# Autodesk Inventor assembly: Grupo_cortadora_MIR
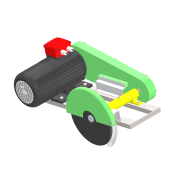
[picture p0: Inventor's stored thumbnail of the model, 180x180]
Saved by Autodesk Inventor 2021 (Build 250183000, 183)
## iProperties
Created: 2021-04-30
Part Number: Grupo_cortadora_MIR
Document SubType Name: Assembly
Designer: maaro
Sending System: Autodesk Translation Framework
Major Version: 7.0
Minor Version: 0.0
Format Version: 0.0
Product Id: Autodesk Translation Framework
Author: Admin
## Documents named in this file (84)
- C:\Users\maaro\Documents\UNAL\Automatización de Procesos de Manufactura\Github\Proyecto_APM\CADs estaciones a automatizar\Estación corte\Grupo_cortadora_MIR.iam
- C:\Users\maaro\Documents\UNAL\Automatización de Procesos de Manufactura\Github\Proyecto_APM\CADs estaciones a automatizar\Estación corte\Grupo_cortadora_MIR.ipt
- C:\Users\maaro\Documents\UNAL\Automatización de Procesos de Manufactura\Github\Proyecto_APM\CADs estaciones a automatizar\Estación corte\Grupo_cortadora_1_MIR.ipt
- C:\Users\maaro\Documents\UNAL\Automatización de Procesos de Manufactura\Github\Proyecto_APM\CADs estaciones a automatizar\Estación corte\Grupo_cortadora_2_MIR.ipt
- C:\Users\maaro\Documents\UNAL\Automatización de Procesos de Manufactura\Github\Proyecto_APM\CADs estaciones a automatizar\Estación corte\Grupo_cortadora_3_MIR.ipt
- C:\Users\maaro\Documents\UNAL\Automatización de Procesos de Manufactura\Github\Proyecto_APM\CADs estaciones a automatizar\Estación corte\Grupo_cortadora_4_MIR.ipt
- C:\Users\maaro\Documents\UNAL\Automatización de Procesos de Manufactura\Github\Proyecto_APM\CADs estaciones a automatizar\Estación corte\Grupo_cortadora_5_MIR.ipt
- C:\Users\maaro\Documents\UNAL\Automatización de Procesos de Manufactura\Github\Proyecto_APM\CADs estaciones a automatizar\Estación corte\Grupo_cortadora_6_MIR.ipt
- C:\Users\maaro\Documents\UNAL\Automatización de Procesos de Manufactura\Github\Proyecto_APM\CADs estaciones a automatizar\Estación corte\Grupo_cortadora_7_MIR.ipt
- C:\Users\maaro\Documents\UNAL\Automatización de Procesos de Manufactura\Github\Proyecto_APM\CADs estaciones a automatizar\Estación corte\Grupo_cortadora_8_MIR.ipt
- C:\Users\maaro\Documents\UNAL\Automatización de Procesos de Manufactura\Github\Proyecto_APM\CADs estaciones a automatizar\Estación corte\Grupo_cortadora_9_MIR.ipt
- C:\Users\maaro\Documents\UNAL\Automatización de Procesos de Manufactura\Github\Proyecto_APM\CADs estaciones a automatizar\Estación corte\Grupo_cortadora_10_MIR.ipt
- C:\Users\maaro\Documents\UNAL\Automatización de Procesos de Manufactura\Github\Proyecto_APM\CADs estaciones a automatizar\Estación corte\Grupo_cortadora_11_MIR.ipt
- C:\Users\maaro\Documents\UNAL\Automatización de Procesos de Manufactura\Github\Proyecto_APM\CADs estaciones a automatizar\Estación corte\Grupo_cortadora_12_MIR.ipt
- C:\Users\maaro\Documents\UNAL\Automatización de Procesos de Manufactura\Github\Proyecto_APM\CADs estaciones a automatizar\Estación corte\Grupo_cortadora_13_MIR.ipt
- C:\Users\maaro\Documents\UNAL\Automatización de Procesos de Manufactura\Github\Proyecto_APM\CADs estaciones a automatizar\Estación corte\Grupo_cortadora_17_MIR.ipt
- C:\Users\maaro\Documents\UNAL\Automatización de Procesos de Manufactura\Github\Proyecto_APM\CADs estaciones a automatizar\Estación corte\Grupo_cortadora_18_MIR.ipt
- C:\Users\maaro\Documents\UNAL\Automatización de Procesos de Manufactura\Github\Proyecto_APM\CADs estaciones a automatizar\Estación corte\Grupo_cortadora_20_MIR.ipt
- C:\Users\maaro\Documents\UNAL\Automatización de Procesos de Manufactura\Github\Proyecto_APM\CADs estaciones a automatizar\Estación corte\Grupo_cortadora_21_MIR.ipt
- C:\Users\maaro\Documents\UNAL\Automatización de Procesos de Manufactura\Github\Proyecto_APM\CADs estaciones a automatizar\Estación corte\Grupo_cortadora_22_MIR.ipt
- C:\Users\maaro\Documents\UNAL\Automatización de Procesos de Manufactura\Github\Proyecto_APM\CADs estaciones a automatizar\Estación corte\Grupo_cortadora_23_MIR.ipt
- C:\Users\maaro\Documents\UNAL\Automatización de Procesos de Manufactura\Github\Proyecto_APM\CADs estaciones a automatizar\Estación corte\Grupo_cortadora_24_MIR.ipt
- C:\Users\maaro\Documents\UNAL\Automatización de Procesos de Manufactura\Github\Proyecto_APM\CADs estaciones a automatizar\Estación corte\Grupo_cortadora_25_MIR.ipt
- C:\Users\maaro\Documents\UNAL\Automatización de Procesos de Manufactura\Github\Proyecto_APM\CADs estaciones a automatizar\Estación corte\Grupo_cortadora_26_MIR.ipt
- C:\Users\maaro\Documents\UNAL\Automatización de Procesos de Manufactura\Github\Proyecto_APM\CADs estaciones a automatizar\Estación corte\Grupo_cortadora_27_MIR.ipt
- C:\Users\maaro\Documents\UNAL\Automatización de Procesos de Manufactura\Github\Proyecto_APM\CADs estaciones a automatizar\Estación corte\Grupo_cortadora_28_MIR.ipt
- C:\Users\maaro\Documents\UNAL\Automatización de Procesos de Manufactura\Github\Proyecto_APM\CADs estaciones a automatizar\Estación corte\Grupo_cortadora_29_MIR.ipt
- C:\Users\maaro\Documents\UNAL\Automatización de Procesos de Manufactura\Github\Proyecto_APM\CADs estaciones a automatizar\Estación corte\Grupo_cortadora_30_MIR.ipt
- C:\Users\maaro\Documents\UNAL\Automatización de Procesos de Manufactura\Github\Proyecto_APM\CADs estaciones a automatizar\Estación corte\Grupo_cortadora_31_MIR.ipt
- C:\Users\maaro\Documents\UNAL\Automatización de Procesos de Manufactura\Github\Proyecto_APM\CADs estaciones a automatizar\Estación corte\Grupo_cortadora_32_MIR.ipt
- C:\Users\maaro\Documents\UNAL\Automatización de Procesos de Manufactura\Github\Proyecto_APM\CADs estaciones a automatizar\Estación corte\Grupo_cortadora_33_MIR.ipt
- C:\Users\maaro\Documents\UNAL\Automatización de Procesos de Manufactura\Github\Proyecto_APM\CADs estaciones a automatizar\Estación corte\Grupo_cortadora_34_MIR.ipt
- C:\Users\maaro\Documents\UNAL\Automatización de Procesos de Manufactura\Github\Proyecto_APM\CADs estaciones a automatizar\Estación corte\Grupo_cortadora_35_MIR.ipt
- C:\Users\maaro\Documents\UNAL\Automatización de Procesos de Manufactura\Github\Proyecto_APM\CADs estaciones a automatizar\Estación corte\Grupo_cortadora_36_MIR.ipt
- C:\Users\maaro\Documents\UNAL\Automatización de Procesos de Manufactura\Github\Proyecto_APM\CADs estaciones a automatizar\Estación corte\Grupo_cortadora_37_MIR.ipt
- C:\Users\maaro\Documents\UNAL\Automatización de Procesos de Manufactura\Github\Proyecto_APM\CADs estaciones a automatizar\Estación corte\Grupo_cortadora_38_MIR.ipt
- C:\Users\maaro\Documents\UNAL\Automatización de Procesos de Manufactura\Github\Proyecto_APM\CADs estaciones a automatizar\Estación corte\Grupo_cortadora_39_MIR.ipt
- C:\Users\maaro\Documents\UNAL\Automatización de Procesos de Manufactura\Github\Proyecto_APM\CADs estaciones a automatizar\Estación corte\Grupo_cortadora_40_MIR.ipt
- C:\Users\maaro\Documents\UNAL\Automatización de Procesos de Manufactura\Github\Proyecto_APM\CADs estaciones a automatizar\Estación corte\Grupo_cortadora_41_MIR.ipt
- C:\Users\maaro\Documents\UNAL\Automatización de Procesos de Manufactura\Github\Proyecto_APM\CADs estaciones a automatizar\Estación corte\Grupo_cortadora_42_MIR.ipt
- C:\Users\maaro\Documents\UNAL\Automatización de Procesos de Manufactura\Github\Proyecto_APM\CADs estaciones a automatizar\Estación corte\Grupo_cortadora_43_MIR.ipt
- C:\Users\maaro\Documents\UNAL\Automatización de Procesos de Manufactura\Github\Proyecto_APM\CADs estaciones a automatizar\Estación corte\Grupo_cortadora_44_MIR.ipt
- C:\Users\maaro\Documents\UNAL\Automatización de Procesos de Manufactura\Github\Proyecto_APM\CADs estaciones a automatizar\Estación corte\Grupo_cortadora_45_MIR.ipt
- C:\Users\maaro\Documents\UNAL\Automatización de Procesos de Manufactura\Github\Proyecto_APM\CADs estaciones a automatizar\Estación corte\Grupo_cortadora_46_MIR.ipt
- C:\Users\maaro\Documents\UNAL\Automatización de Procesos de Manufactura\Github\Proyecto_APM\CADs estaciones a automatizar\Estación corte\Grupo_cortadora_47_MIR.ipt
- C:\Users\maaro\Documents\UNAL\Automatización de Procesos de Manufactura\Github\Proyecto_APM\CADs estaciones a automatizar\Estación corte\Grupo_cortadora_48_MIR.ipt
- C:\Users\maaro\Documents\UNAL\Automatización de Procesos de Manufactura\Github\Proyecto_APM\CADs estaciones a automatizar\Estación corte\Grupo_cortadora_49_MIR.ipt
- C:\Users\maaro\Documents\UNAL\Automatización de Procesos de Manufactura\Github\Proyecto_APM\CADs estaciones a automatizar\Estación corte\Grupo_cortadora_50_MIR.ipt
- C:\Users\maaro\Documents\UNAL\Automatización de Procesos de Manufactura\Github\Proyecto_APM\CADs estaciones a automatizar\Estación corte\Grupo_cortadora_51_MIR.ipt
- C:\Users\maaro\Documents\UNAL\Automatización de Procesos de Manufactura\Github\Proyecto_APM\CADs estaciones a automatizar\Estación corte\Grupo_cortadora_52_MIR.ipt
- C:\Users\maaro\Documents\UNAL\Automatización de Procesos de Manufactura\Github\Proyecto_APM\CADs estaciones a automatizar\Estación corte\Grupo_cortadora_53_MIR.ipt
- C:\Users\maaro\Documents\UNAL\Automatización de Procesos de Manufactura\Github\Proyecto_APM\CADs estaciones a automatizar\Estación corte\Grupo_cortadora_54_MIR.ipt
- C:\Users\maaro\Documents\UNAL\Automatización de Procesos de Manufactura\Github\Proyecto_APM\CADs estaciones a automatizar\Estación corte\Grupo_cortadora_55_MIR.ipt
- C:\Users\maaro\Documents\UNAL\Automatización de Procesos de Manufactura\Github\Proyecto_APM\CADs estaciones a automatizar\Estación corte\Grupo_cortadora_56_MIR.ipt
- C:\Users\maaro\Documents\UNAL\Automatización de Procesos de Manufactura\Github\Proyecto_APM\CADs estaciones a automatizar\Estación corte\Grupo_cortadora_57_MIR.ipt
- C:\Users\maaro\Documents\UNAL\Automatización de Procesos de Manufactura\Github\Proyecto_APM\CADs estaciones a automatizar\Estación corte\Grupo_cortadora_58_MIR.ipt
- C:\Users\maaro\Documents\UNAL\Automatización de Procesos de Manufactura\Github\Proyecto_APM\CADs estaciones a automatizar\Estación corte\Grupo_cortadora_59_MIR.ipt
- C:\Users\maaro\Documents\UNAL\Automatización de Procesos de Manufactura\Github\Proyecto_APM\CADs estaciones a automatizar\Estación corte\Grupo_cortadora_60_MIR.ipt
- C:\Users\maaro\Documents\UNAL\Automatización de Procesos de Manufactura\Github\Proyecto_APM\CADs estaciones a automatizar\Estación corte\Grupo_cortadora_61_MIR.ipt
- C:\Users\maaro\Documents\UNAL\Automatización de Procesos de Manufactura\Github\Proyecto_APM\CADs estaciones a automatizar\Estación corte\Grupo_cortadora_62_MIR.ipt
- C:\Users\maaro\Documents\UNAL\Automatización de Procesos de Manufactura\Github\Proyecto_APM\CADs estaciones a automatizar\Estación corte\Grupo_cortadora_63_MIR.ipt
- C:\Users\maaro\Documents\UNAL\Automatización de Procesos de Manufactura\Github\Proyecto_APM\CADs estaciones a automatizar\Estación corte\Grupo_cortadora_64_MIR.ipt
- C:\Users\maaro\Documents\UNAL\Automatización de Procesos de Manufactura\Github\Proyecto_APM\CADs estaciones a automatizar\Estación corte\Grupo_cortadora_65_MIR.ipt
- C:\Users\maaro\Documents\UNAL\Automatización de Procesos de Manufactura\Github\Proyecto_APM\CADs estaciones a automatizar\Estación corte\Grupo_cortadora_66_MIR.ipt
- C:\Users\maaro\Documents\UNAL\Automatización de Procesos de Manufactura\Github\Proyecto_APM\CADs estaciones a automatizar\Estación corte\Grupo_cortadora_67_MIR.ipt
- C:\Users\maaro\Documents\UNAL\Automatización de Procesos de Manufactura\Github\Proyecto_APM\CADs estaciones a automatizar\Estación corte\Grupo_cortadora_68_MIR.ipt
- C:\Users\maaro\Documents\UNAL\Automatización de Procesos de Manufactura\Github\Proyecto_APM\CADs estaciones a automatizar\Estación corte\Grupo_cortadora_69_MIR.ipt
- C:\Users\maaro\Documents\UNAL\Automatización de Procesos de Manufactura\Github\Proyecto_APM\CADs estaciones a automatizar\Estación corte\Grupo_cortadora_70_MIR.ipt
- C:\Users\maaro\Documents\UNAL\Automatización de Procesos de Manufactura\Github\Proyecto_APM\CADs estaciones a automatizar\Estación corte\Grupo_cortadora_71_MIR.ipt
- C:\Users\maaro\Documents\UNAL\Automatización de Procesos de Manufactura\Github\Proyecto_APM\CADs estaciones a automatizar\Estación corte\Grupo_cortadora_72_MIR.ipt
- C:\Users\maaro\Documents\UNAL\Automatización de Procesos de Manufactura\Github\Proyecto_APM\CADs estaciones a automatizar\Estación corte\Grupo_cortadora_73_MIR.ipt
- C:\Users\maaro\Documents\UNAL\Automatización de Procesos de Manufactura\Github\Proyecto_APM\CADs estaciones a automatizar\Estación corte\Grupo_cortadora_74_MIR.ipt
- C:\Users\maaro\Documents\UNAL\Automatización de Procesos de Manufactura\Github\Proyecto_APM\CADs estaciones a automatizar\Estación corte\Grupo_cortadora_75_MIR.ipt
- C:\Users\maaro\Documents\UNAL\Automatización de Procesos de Manufactura\Github\Proyecto_APM\CADs estaciones a automatizar\Estación corte\Grupo_cortadora_76_MIR.ipt
- C:\Users\maaro\Documents\UNAL\Automatización de Procesos de Manufactura\Github\Proyecto_APM\CADs estaciones a automatizar\Estación corte\Grupo_cortadora_77_MIR.ipt
- C:\Users\maaro\Documents\UNAL\Automatización de Procesos de Manufactura\Github\Proyecto_APM\CADs estaciones a automatizar\Estación corte\Grupo_cortadora_78_MIR.ipt
- C:\Users\maaro\Documents\UNAL\Automatización de Procesos de Manufactura\Github\Proyecto_APM\CADs estaciones a automatizar\Estación corte\Grupo_cortadora_79_MIR.ipt
- C:\Users\maaro\Documents\UNAL\Automatización de Procesos de Manufactura\Github\Proyecto_APM\CADs estaciones a automatizar\Estación corte\Grupo_cortadora_80_MIR.ipt
- C:\Users\maaro\Documents\UNAL\Automatización de Procesos de Manufactura\Github\Proyecto_APM\CADs estaciones a automatizar\Estación corte\Grupo_cortadora_81_MIR.ipt
- C:\Users\maaro\Documents\UNAL\Automatización de Procesos de Manufactura\Github\Proyecto_APM\CADs estaciones a automatizar\Estación corte\Grupo_cortadora_82_MIR.ipt
- C:\Users\maaro\Documents\UNAL\Automatización de Procesos de Manufactura\Github\Proyecto_APM\CADs estaciones a automatizar\Estación corte\Grupo_cortadora_83_MIR.ipt
- C:\Users\maaro\Documents\UNAL\Automatización de Procesos de Manufactura\Github\Proyecto_APM\CADs estaciones a automatizar\Estación corte\Grupo_cortadora_84_MIR.ipt
- C:\Users\maaro\Documents\UNAL\Automatización de Procesos de Manufactura\Github\Proyecto_APM\CADs estaciones a automatizar\Estación corte\Protector.ipt
- C:\Users\maaro\Documents\Inventor\Content Center Files\R2021\en-US\DIN 920\DIN 920 - M5 x 5.ipt
## Components (84 placed, 83 different names)
1. Grupo_cortadora_MIR:1
2. Grupo_cortadora_1_MIR:1
3. Grupo_cortadora_2_MIR:1
4. Grupo_cortadora_3_MIR:1
5. Grupo_cortadora_4_MIR:1
6. Grupo_cortadora_5_MIR:1
7. Grupo_cortadora_6_MIR:1
8. Grupo_cortadora_7_MIR:1
9. Grupo_cortadora_8_MIR:1
10. Grupo_cortadora_9_MIR:1
11. Grupo_cortadora_10_MIR:1
12. Grupo_cortadora_11_MIR:1
13. Grupo_cortadora_12_MIR:1
14. Grupo_cortadora_13_MIR:1
15. Grupo_cortadora_17_MIR:1
16. Grupo_cortadora_18_MIR:1
17. Grupo_cortadora_20_MIR:1
18. Grupo_cortadora_21_MIR:1
19. Grupo_cortadora_22_MIR:1
20. Grupo_cortadora_23_MIR:1
21. Grupo_cortadora_24_MIR:1
22. Grupo_cortadora_25_MIR:1
23. Grupo_cortadora_26_MIR:1
24. Grupo_cortadora_27_MIR:1
25. Grupo_cortadora_28_MIR:1
26. Grupo_cortadora_29_MIR:1
27. Grupo_cortadora_30_MIR:1
28. Grupo_cortadora_31_MIR:1
29. Grupo_cortadora_32_MIR:1
30. Grupo_cortadora_33_MIR:1
31. Grupo_cortadora_34_MIR:1
32. Grupo_cortadora_35_MIR:1
33. Grupo_cortadora_36_MIR:1
34. Grupo_cortadora_37_MIR:1
35. Grupo_cortadora_38_MIR:1
36. Grupo_cortadora_39_MIR:1
37. Grupo_cortadora_40_MIR:1
38. Grupo_cortadora_41_MIR:1
39. Grupo_cortadora_42_MIR:1
40. Grupo_cortadora_43_MIR:1
41. Grupo_cortadora_44_MIR:1
42. Grupo_cortadora_45_MIR:1
43. Grupo_cortadora_46_MIR:1
44. Grupo_cortadora_47_MIR:1
45. Grupo_cortadora_48_MIR:1
46. Grupo_cortadora_49_MIR:1
47. Grupo_cortadora_50_MIR:1
48. Grupo_cortadora_51_MIR:1
49. Grupo_cortadora_52_MIR:1
50. Grupo_cortadora_53_MIR:1
51. Grupo_cortadora_54_MIR:1
52. Grupo_cortadora_55_MIR:1
53. Grupo_cortadora_56_MIR:1
54. Grupo_cortadora_57_MIR:1
55. Grupo_cortadora_58_MIR:1
56. Grupo_cortadora_59_MIR:1
57. Grupo_cortadora_60_MIR:1
58. Grupo_cortadora_61_MIR:1
59. Grupo_cortadora_62_MIR:1
60. Grupo_cortadora_63_MIR:1
61. Grupo_cortadora_64_MIR:1
62. Grupo_cortadora_65_MIR:1
63. Grupo_cortadora_66_MIR:1
64. Grupo_cortadora_67_MIR:1
65. Grupo_cortadora_68_MIR:1 — Flush:1, Flush:2
66. Grupo_cortadora_69_MIR:1
67. Grupo_cortadora_70_MIR:1
68. Grupo_cortadora_71_MIR:1
69. Grupo_cortadora_72_MIR:1
70. Grupo_cortadora_73_MIR:1
71. Grupo_cortadora_74_MIR:1
72. Grupo_cortadora_75_MIR:1
73. Grupo_cortadora_76_MIR:1
74. Grupo_cortadora_77_MIR:1
75. Grupo_cortadora_78_MIR:1
76. Grupo_cortadora_79_MIR:1
77. Grupo_cortadora_80_MIR:1
78. Grupo_cortadora_81_MIR:1
79. Grupo_cortadora_82_MIR:1
80. Grupo_cortadora_83_MIR:1
81. Grupo_cortadora_84_MIR:1
82. Protector:1 — Flush:1, Flush:2, Insert:1, Insert:2
83. DIN 920 M5 x 5:1 — Insert:1
84. DIN 920 M5 x 5:2 — Insert:2
## Relationships (4: Flush 2, Insert 2)
- Flush:1: Grupo_cortadora_68_MIR:1 ↔ Protector:1
- Flush:2: Grupo_cortadora_68_MIR:1 ↔ Protector:1
- Insert:1: Protector:1 ↔ DIN 920 M5 x 5:1
- Insert:2: Protector:1 ↔ DIN 920 M5 x 5:2
